# Autodesk Inventor assembly: capistan
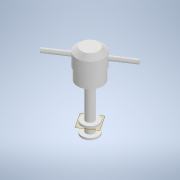
[picture p0: Inventor's stored thumbnail of the model, 180x180]
Saved by Autodesk Inventor 2020.2 (Build 242310000, 310)
## iProperties
Created: 2021-01-29
Part Number: capistan
Document SubType Name: Assembly
Designer: con_c_000
Author: con_c_000
## Documents named in this file (3)
- C:\Users\con_c_000\Documents\Inventor\Content Center Files\FIRST ROBOT\capistan.iam
- C:\Users\con_c_000\Documents\Inventor\Content Center Files\FIRST ROBOT\capistan lower.ipt
- C:\Users\con_c_000\Documents\Inventor\Content Center Files\FIRST ROBOT\capistan upper.ipt
## Components (2 placed, 2 different names)
1. capistan lower:1 — Rotational:1
2. capistan upper:1 — Rotational:1
## Relationships (1: RevoluteJoint 1)
- Rotational:1 [RevoluteJoint]: capistan lower:1 ↔ capistan upper:1
